# Autodesk Inventor assembly: assy_mission_traffic_light
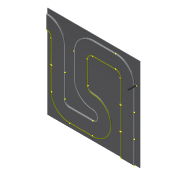
[picture p0: Inventor's stored thumbnail of the model, 180x180]
Saved by Autodesk Inventor 2018 (Build 220112000, 112)
## iProperties
Created: 2017-11-13
Part Number: assy_mission_traffic_light
Document SubType Name: Assembly
Designer: Platform
Author: Platform
## Documents named in this file (6)
- C:\Users\Platform\Desktop\autorace_track\track_model\autorace_rbizchallenge2017\assembled\assy_mission_traffic_light.iam
- C:\Users\Platform\Desktop\autorace_track\track_model\autorace_rbizchallenge2017\assembled\assy_lower_plates.iam
- C:\Users\Platform\Desktop\autorace_track\track_model\autorace_rbizchallenge2017\assembled\assy_straight.iam
- C:\Users\Platform\Desktop\autorace_track\track_model\autorace_rbizchallenge2017\assembled\assy_curved_left.iam
- C:\Users\Platform\Desktop\autorace_track\track_model\autorace_rbizchallenge2017\assembled\assy_curved_right.iam
- C:\Users\Platform\Desktop\autorace_track\track_model\autorace_rbizchallenge2017\parts\ipt\trafficlight.ipt
## Components (17 placed, 5 different names)
1. assy_lower_plates:1 [sub-assembly] — Mate:1, Flush:1, Flush:2, Mate:2, Mate:4, Mate:6, Mate:9, Mate:12, Mate:15, Mate:18, Mate:21, Mate:24, Mate:27, Mate:30, Mate:33, Mate:36, Mate:38, Mate:41, Mate:43
2. assy_straight:1 [sub-assembly] — Mate:1, Flush:1, Flush:2, Flush:3, Mate:3
3. assy_straight:2 [sub-assembly] — Mate:2, Flush:3, Mate:3, Mate:5, Flush:4, Mate:42
4. assy_straight:3 [sub-assembly] — Mate:4, Mate:5, Flush:4, Mate:7, Mate:8
5. assy_curved_left:1 [sub-assembly] — Mate:6, Mate:7, Mate:8, Mate:10, Mate:11
6. assy_straight:4 [sub-assembly] — Mate:9, Mate:10, Mate:11, Mate:13, Mate:14
7. assy_curved_left:2 [sub-assembly] — Mate:12, Mate:13, Mate:14, Mate:16, Mate:17
8. assy_straight:5 [sub-assembly] — Mate:15, Mate:16, Mate:17, Mate:19, Mate:20
9. assy_curved_left:3 [sub-assembly] — Mate:38, Mate:39, Mate:40
10. assy_curved_left:4 [sub-assembly] — Mate:18, Mate:19, Mate:20, Mate:22, Mate:23
11. assy_curved_right:1 [sub-assembly] — Mate:21, Mate:22, Mate:23, Mate:25, Mate:26
12. assy_curved_right:2 [sub-assembly] — Mate:24, Mate:25, Mate:26, Mate:28, Mate:29
13. assy_straight:6 [sub-assembly] — Mate:27, Mate:28, Mate:29, Mate:31, Mate:32
14. assy_curved_right:3 [sub-assembly] — Mate:30, Mate:31, Mate:32, Mate:34, Mate:35
15. assy_straight:7 [sub-assembly] — Mate:33, Mate:34, Mate:35, Flush:5, Mate:37
16. assy_straight:8 [sub-assembly] — Mate:36, Flush:5, Mate:37, Mate:39, Mate:40
17. trafficlight:1 — Mate:41, Mate:42, Mate:43
## Relationships (48: Mate 43, Flush 5)
- Mate:1: assy_lower_plates:1 ↔ assy_straight:1
- Flush:1: assy_lower_plates:1 ↔ assy_straight:1
- Flush:2 (100 mm): assy_lower_plates:1 ↔ assy_straight:1
- Mate:2: assy_lower_plates:1 ↔ assy_straight:2
- Flush:3: assy_straight:1 ↔ assy_straight:2
- Mate:3: assy_straight:1 ↔ assy_straight:2
- Mate:4: assy_lower_plates:1 ↔ assy_straight:3
- Mate:5: assy_straight:2 ↔ assy_straight:3
- Flush:4: assy_straight:2 ↔ assy_straight:3
- Mate:6: assy_lower_plates:1 ↔ assy_curved_left:1
- Mate:7: assy_straight:3 ↔ assy_curved_left:1
- Mate:8: assy_straight:3 ↔ assy_curved_left:1
- Mate:9: assy_lower_plates:1 ↔ assy_straight:4
- Mate:10: assy_curved_left:1 ↔ assy_straight:4
- Mate:11: assy_curved_left:1 ↔ assy_straight:4
- Mate:12: assy_lower_plates:1 ↔ assy_curved_left:2
- Mate:13: assy_straight:4 ↔ assy_curved_left:2
- Mate:14: assy_straight:4 ↔ assy_curved_left:2
- Mate:15: assy_lower_plates:1 ↔ assy_straight:5
- Mate:16: assy_curved_left:2 ↔ assy_straight:5
- Mate:17: assy_curved_left:2 ↔ assy_straight:5
- Mate:18: assy_lower_plates:1 ↔ assy_curved_left:4
- Mate:19: assy_straight:5 ↔ assy_curved_left:4
- Mate:20: assy_straight:5 ↔ assy_curved_left:4
- Mate:21: assy_lower_plates:1 ↔ assy_curved_right:1
- Mate:22: assy_curved_left:4 ↔ assy_curved_right:1
- Mate:23: assy_curved_left:4 ↔ assy_curved_right:1
- Mate:24: assy_lower_plates:1 ↔ assy_curved_right:2
- Mate:25: assy_curved_right:1 ↔ assy_curved_right:2
- Mate:26: assy_curved_right:1 ↔ assy_curved_right:2
- Mate:27: assy_lower_plates:1 ↔ assy_straight:6
- Mate:28: assy_curved_right:2 ↔ assy_straight:6
- Mate:29: assy_curved_right:2 ↔ assy_straight:6
- Mate:30: assy_lower_plates:1 ↔ assy_curved_right:3
- Mate:31: assy_straight:6 ↔ assy_curved_right:3
- Mate:32: assy_straight:6 ↔ assy_curved_right:3
- Mate:33: assy_lower_plates:1 ↔ assy_straight:7
- Mate:34: assy_curved_right:3 ↔ assy_straight:7
- Mate:35: assy_curved_right:3 ↔ assy_straight:7
- Mate:36: assy_lower_plates:1 ↔ assy_straight:8
- Flush:5: assy_straight:7 ↔ assy_straight:8
- Mate:37: assy_straight:7 ↔ assy_straight:8
- Mate:38: assy_lower_plates:1 ↔ assy_curved_left:3
- Mate:39: assy_curved_left:3 ↔ assy_straight:8
- Mate:40: assy_curved_left:3 ↔ assy_straight:8
- Mate:41: assy_lower_plates:1 ↔ trafficlight:1
- Mate:42: assy_straight:2 ↔ trafficlight:1
- Mate:43 (-500 mm): assy_lower_plates:1 ↔ trafficlight:1
